# Autodesk Inventor assembly: Povorot_mec.ipt
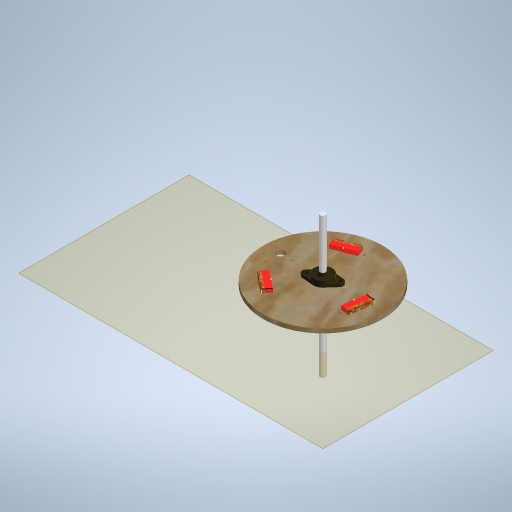
[picture p0: Inventor's stored thumbnail of the model, 512x512]
Saved by Autodesk Inventor 2023.1 (Build 271208000, 208)
## iProperties
Created: 2023-12-24
Part Number: Povorot_mec.ipt
Document SubType Name: Assembly
Designer: Dell
Author: Dell
## Documents named in this file (15)
- C:\Users\Dell\Desktop\Ворона и Лисица\Povorot_mec.ipt.iam
- C:\Users\Dell\Downloads\Pitsco Education-739085.ipt
- C:\Users\Dell\Desktop\Ворона и Лисица\Cap_pipes.ipt
- C:\Users\Dell\Downloads\Pitsco Education-739028.ipt
- C:\Users\Dell\Desktop\Ворона и Лисица\Fanerka.ipt
- C:\Users\Dell\Desktop\Ворона и Лисица\Prostavka.ipt
- C:\Users\Dell\Desktop\Ворона и Лисица\Det_podsh.ipt
- C:\Users\Dell\Desktop\Ворона и Лисица\Podsh.ipt
- C:\Users\Dell\Downloads\User Library-Bearing KFL08.ipt
- C:\Users\Dell\Desktop\Ворона и Лисица\trubka.ipt
- C:\Users\Dell\Downloads\45121 tetrix max torquenado motor pack\45121 TETRIX MAX TorqueNADO Motor Pack\39079_TXM-Motor Shaft Hub With Set Screw.ipt
- C:\Users\Dell\Downloads\SHF8\SHF8 Горизонтальный держатель вала.ipt
- C:\Users\Dell\Documents\Inventor\Content Center Files\R2023\ru-RU\ISO 14583\ISO 14583 — M5x16-4.8.ipt
- C:\Users\Dell\Documents\Inventor\Content Center Files\R2023\ru-RU\ISO 7046-1 H(1)\ISO 7046-1 - M6 x 20_ - 4.8 - H - ISO.ipt
- C:\Users\Dell\Downloads\44260_txm torquenado dc motor.ipt
## Components (22 placed, 14 different names)
1. Pitsco Education-739085:1 — Жесткий:6, Совмещение:10, Совмещение:11, Совмещение:13, Совмещение:16
2. Cap_pipes:1 — Цилиндрический:2, Совмещение:8, Совмещение:9
3. Pitsco Education-739028:1
4. Fanerka:1 — Совмещение:9, Плоский:1, Плоский:2, Плоский:3, С поворотом:3, С поворотом:4, С поворотом:5
5. Prostavka:1 — Цилиндрический:2, Совмещение:8, Жесткий:5
6. User Library-Bearing KFL08:1 — С поворотом:3, С поворотом:4
7. trubka:1 — Жесткий:5, Жесткий:6, Цилиндрический:5
8. 39079_TXM-Motor Shaft Hub With Set Screw:1
9. Винт ISO 14583:2011(E) M5x16-4.8:2
10. Винт ISO 14583:2011(E) M5x16-4.8:3
11. SHF8 Горизонтальный держатель вала:3 — Цилиндрический:5
12. ISO 7046-1 H M6 x 20 - 4.8 - H:1 — Совмещение:10
13. ISO 7046-1 H M6 x 20 - 4.8 - H:2 — Совмещение:11
14. ISO 7046-1 H M6 x 20 - 4.8 - H:3 — Совмещение:13
15. ISO 7046-1 H M6 x 20 - 4.8 - H:4 — Совмещение:16
16. 44260_txm torquenado dc motor:1 — С поворотом:5
17. Det_podsh:2 — С поворотом:1, Плоский:1, Плоский:2, Плоский:3
18. Podsh:1 — С поворотом:1
19. Det_podsh:3
20. Podsh:2
21. Det_podsh:4
22. Podsh:3
## Component patterns: (3 elements, first: Det_podsh:2 + Podsh:1)
## Relationships (17: Mate 6, RevoluteJoint 4, PlanarJoint 3, CylindricalJoint 2, WeldJoint 2)
- Цилиндрический:2 [CylindricalJoint]: Cap_pipes:1 ↔ Prostavka:1
- Совмещение:8 [Mate]: Cap_pipes:1 ↔ Prostavka:1
- Совмещение:9 [Mate]: Cap_pipes:1 ↔ Fanerka:1
- С поворотом:1 [RevoluteJoint]: Det_podsh:2 ↔ Podsh:1
- Плоский:1 [PlanarJoint]: Fanerka:1 ↔ Det_podsh:2
- Плоский:2 [PlanarJoint]: Fanerka:1 ↔ Det_podsh:2
- Плоский:3 [PlanarJoint]: Fanerka:1 ↔ Det_podsh:2
- Жесткий:5 [WeldJoint]: Prostavka:1 ↔ trubka:1
- Жесткий:6 [WeldJoint]: Pitsco Education-739085:1 ↔ trubka:1
- С поворотом:3 [RevoluteJoint]: Fanerka:1 ↔ User Library-Bearing KFL08:1
- С поворотом:4 [RevoluteJoint]: Fanerka:1 ↔ User Library-Bearing KFL08:1
- Цилиндрический:5 [CylindricalJoint]: trubka:1 ↔ SHF8 Горизонтальный держатель вала:3
- Совмещение:10 [Mate]: Pitsco Education-739085:1 ↔ ISO 7046-1 H M6 x 20 - 4.8 - H:1
- Совмещение:11 [Mate]: Pitsco Education-739085:1 ↔ ISO 7046-1 H M6 x 20 - 4.8 - H:2
- Совмещение:13 [Mate]: Pitsco Education-739085:1 ↔ ISO 7046-1 H M6 x 20 - 4.8 - H:3
- Совмещение:16 [Mate]: Pitsco Education-739085:1 ↔ ISO 7046-1 H M6 x 20 - 4.8 - H:4
- С поворотом:5 [RevoluteJoint]: Fanerka:1 ↔ 44260_txm torquenado dc motor:1
